# Autodesk Inventor assembly: quartz window assembly
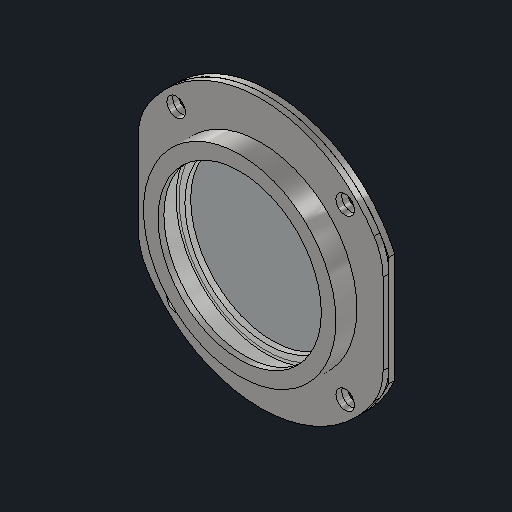
[picture p0: Inventor's stored thumbnail of the model, 512x512]
Saved by Autodesk Inventor 2026 (Build 300175050, 175E)
## iProperties
Created: 2024-05-22
Part Number: quartz window assembly
Document SubType Name: Assembly
Designer: kuzmin
Mass: 22.6702 g
Surface Area: 66.29 cm^2
Volume: 4.58219 cm^3
Density: 4.94746 g/cm^3
Author: kuzmin
## Documents named in this file (5)
- C:\Users\queez\Dropbox\Drawings\PIHTI\Plasma Vessel\Plasma-Box\quartz-window-30mm-in-holder.iam
- C:\Users\queez\Dropbox\Drawings\PIHTI\Plasma Vessel\Plasma-Box\probe-gate-spacer\probe-gate-spacer-quartz-holder.ipt
- C:\Users\queez\Dropbox\Drawings\PIHTI\Plasma Vessel\Plasma-Box\probe-gate-spacer.ipt
- C:\Users\queez\Dropbox\Drawings\PIHTI\Plasma Vessel\Plasma-Box\quartz-disk-window.ipt
- C:\Users\queez\Dropbox\Drawings\PIHTI\Plasma Vessel\Plasma-Box\quartz-disk-window-holder.ipt
## Components (3 placed, 3 different names)
1. probe-gate-spacer-quartz-holder:1 — Mate:5
2. quartz-disk-window:1
3. quartz-disk-window-holder:1 — Mate:5
## Relationships (5: Mate 5)
- [Mate]: probe-gate-spacer-quartz-holder:1 ↔ quartz-disk-window:1
- [Mate]: quartz-disk-window:1 ↔ quartz-disk-window-holder:1
- [Mate]: probe-gate-spacer-quartz-holder:1 ↔ quartz-disk-window-holder:1
- [Mate]: probe-gate-spacer-quartz-holder:1 ↔ quartz-disk-window-holder:1
- Mate:5: probe-gate-spacer-quartz-holder:1 ↔ quartz-disk-window-holder:1
